# Autodesk Inventor assembly: bearing_holder_assembly
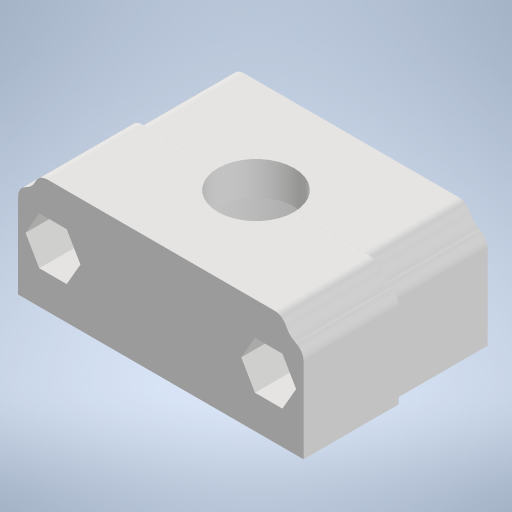
[picture p0: Inventor's stored thumbnail of the model, 512x512]
Saved by Autodesk Inventor 2024 (Build 280153000, 153)
## iProperties
Created: 2024-02-02
Part Number: bearing_holder_assembly
Document SubType Name: Assembly
Designer: Pintu
Author: Pintu
## Documents named in this file (3)
- D:\CMC\my_inventor\ArmBo_v2\bearing_holder_assembly.iam
- D:\CMC\my_inventor\ArmBo_v2\bearing_holder_v3.ipt
- D:\CMC\my_inventor\ArmBo_v2\bearing_holder_top_test_v1.ipt
## Components (2 placed, 2 different names)
1. bearing_holder_v3:1 — Mate:1, Mate:2
2. bearing_holder_top_test_v1:1 — Mate:1, Mate:2
## Relationships (2: Mate 2)
- Mate:1: bearing_holder_v3:1 ↔ bearing_holder_top_test_v1:1
- Mate:2: bearing_holder_v3:1 ↔ bearing_holder_top_test_v1:1
